# Autodesk Inventor assembly: Fr.wing
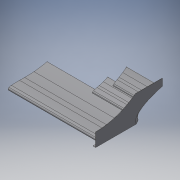
[picture p0: Inventor's stored thumbnail of the model, 180x180]
Saved by Autodesk Inventor 2018.2 (Build 222227000, 227)
## iProperties
Created: 2018-02-26
Part Number: Fr.wing
Material: 一般
Document SubType Name: Assembly
Designer: ku_sk
Author: ku_sk
## Documents named in this file (5)
- C:\Users\ku_sk\Documents\Inventor\AeroCAD2018\設計\Fr.wing\Fr.wing.iam
- C:\Users\ku_sk\Documents\Inventor\AeroCAD2018\設計\Fr.wing\parts\endplate.ipt
- C:\Users\ku_sk\Documents\Inventor\AeroCAD2018\設計\Fr.wing\parts\mainflap.ipt
- C:\Users\ku_sk\Documents\Inventor\AeroCAD2018\設計\Fr.wing\parts\subflap.ipt
- C:\Users\ku_sk\Documents\Inventor\AeroCAD2018\設計\Fr.wing\parts\subflap2.ipt
## Components (4 placed, 4 different names)
1. endplate:1 — メイト:1, メイト:2, メイト:4, メイト:5
2. mainflap:1 — メイト:2, 角度:1
3. subflap2:1 — メイト:5, 角度:1, 角度:2
4. subflap:2 — メイト:4, 角度:2
## Relationships (6: Mate 4, Angle 2)
- メイト:1 [Mate]: endplate:1
- メイト:2 [Mate]: endplate:1 ↔ mainflap:1
- メイト:4 [Mate]: endplate:1 ↔ subflap:2
- メイト:5 [Mate]: endplate:1 ↔ subflap2:1
- 角度:1 [Angle] (-15 deg): mainflap:1 ↔ subflap2:1
- 角度:2 [Angle] (-15 deg): subflap2:1 ↔ subflap:2
